# Autodesk Inventor assembly: KillSwitchAssembly
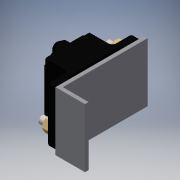
[picture p0: Inventor's stored thumbnail of the model, 180x180]
Saved by Autodesk Inventor 2017 (Build 210142000, 142)
## iProperties
Created: 2020-02-29
Part Number: KillSwitchAssembly
Document SubType Name: Assembly
Designer: S338674153
Author: S338674153
## Documents named in this file (3)
- \\ad.ocdsb.ca\studenthome\3\S338674153\FRC 2020\FullRobotRefactor\Parts\KillSwitchAssembly.iam
- \\ad.ocdsb.ca\studenthome\3\S338674153\FRC 2020\FullRobotRefactor\Parts\KillSwitchSupport.ipt
- \\ad.ocdsb.ca\studenthome\3\S338674153\FRC 2020\FullRobotRefactor\Parts\am-0282 120a Circuit Breaker.ipt
## Components (2 placed, 2 different names)
1. KillSwitchSupport:1 — Mate:1, Flush:1, Flush:2
2. am-0282 120a Circuit Breaker:1 — Mate:1, Flush:1, Flush:2
## Relationships (3: Flush 2, Mate 1)
- Mate:1: KillSwitchSupport:1 ↔ am-0282 120a Circuit Breaker:1
- Flush:1: KillSwitchSupport:1 ↔ am-0282 120a Circuit Breaker:1
- Flush:2 (-2.54 mm): KillSwitchSupport:1 ↔ am-0282 120a Circuit Breaker:1
